# Autodesk Inventor assembly: McCrea_final_scene_walle
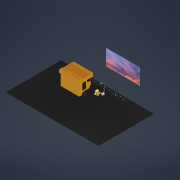
[picture p0: Inventor's stored thumbnail of the model, 180x180]
Saved by Autodesk Inventor 2022 (Build 260153000, 153)
## iProperties
Created: 2022-02-01
Part Number: McCrea_final_scene_walle
Document SubType Name: Assembly
Designer: MatusBarany
Author: MatusBarany
## Documents named in this file (8)
- C:\Users\MatusBarany\Documents\Inventor\wall-e\assembly\McCrea_final_scene_walle.iam
- C:\Users\MatusBarany\Documents\Inventor\wall-e\matus\bench\McCrea_assembly_walle.iam
- C:\Users\MatusBarany\Documents\Inventor\wall-e\assembly\McCrea_WALLE_bez_HEAD_walle.iam
- C:\Users\MatusBarany\Documents\Inventor\wall-e\matus\lampa\McCrea_lampa_walle.ipt
- C:\Users\MatusBarany\Documents\Inventor\wall-e\lukas\McCrea_Plot_walle.ipt
- C:\Users\MatusBarany\Documents\Inventor\wall-e\matus\plocha\McCrea_plocha_walle.ipt
- C:\Users\MatusBarany\Documents\Inventor\wall-e\assembly\background.ipt
- C:\Users\MatusBarany\Documents\Inventor\wall-e\assembly\McCrea_car_walle.iam
## Components (10 placed, 7 different names)
1. McCrea_assembly_walle:1 [sub-assembly]
2. McCrea_WALLE_bez_HEAD_walle:1 [sub-assembly]
3. McCrea_lampa_walle:1 — Mate:4
4. McCrea_plocha_walle:1 — Mate:4, Mate:5, Mate:6, Mate:7
5. McCrea_Plot_walle:2
6. background:1
7. McCrea_Plot_walle:3 — Mate:5
8. McCrea_Plot_walle:4 — Mate:6
9. McCrea_Plot_walle:5 — Mate:7
10. McCrea_car_walle:1 [sub-assembly]
## Relationships (4: Mate 4)
- Mate:4: McCrea_lampa_walle:1 ↔ McCrea_plocha_walle:1
- Mate:5: McCrea_plocha_walle:1 ↔ McCrea_Plot_walle:3
- Mate:6: McCrea_plocha_walle:1 ↔ McCrea_Plot_walle:4
- Mate:7: McCrea_plocha_walle:1 ↔ McCrea_Plot_walle:5
